# Autodesk Inventor assembly: Робот
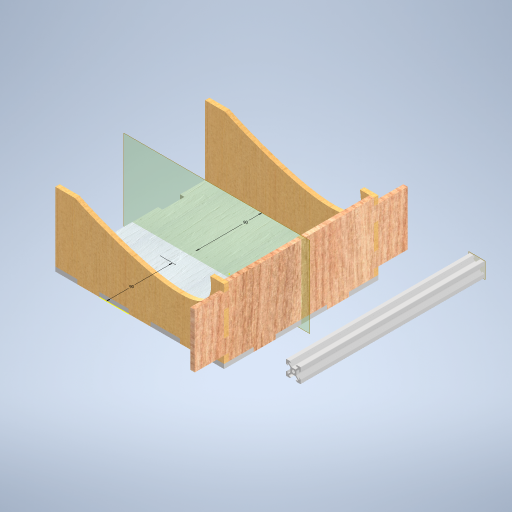
[picture p0: Inventor's stored thumbnail of the model, 512x512]
Saved by Autodesk Inventor 2024.2 (Build 282272000, 272)
## iProperties
Created: 2026-01-27
Part Number: Робот
Document SubType Name: Assembly
Designer: Service
Author: Service
## Documents named in this file (5)
- C:\Users\Zakhar\Documents\Artist-v2\3D\Робот.iam
- C:\Users\Zakhar\Documents\Artist-v2\3D\Низ робота.ipt
- C:\Users\Zakhar\Documents\Artist-v2\3D\бок.ipt
- C:\Users\Zakhar\Documents\Artist-v2\3D\перед.ipt
- C:\Users\Zakhar\Documents\Artist-v2\3D\в_профиль 2020.ipt
## Components (5 placed, 4 different names)
1. Низ робота:1 — Заподлицо:1, Совмещение:1, Заподлицо:2, Симметрия:1, Совмещение:2, Заподлицо:3, Заподлицо:4, Совмещение:3, Заподлицо:5
2. бок:1 — Заподлицо:1, Совмещение:1, Заподлицо:2, Симметрия:1
3. бок:2 — Совмещение:2, Заподлицо:3, Заподлицо:4
4. перед:1 — Совмещение:3, Заподлицо:5
5. в_профиль 2020:1
## Relationships (9: Flush 5, Mate 3, Symmetry 1)
- Заподлицо:1 [Flush]: Низ робота:1 ↔ бок:1
- Совмещение:1 [Mate]: Низ робота:1 ↔ бок:1
- Заподлицо:2 [Flush]: Низ робота:1 ↔ бок:1
- Симметрия:1 [Symmetry]: Низ робота:1 ↔ бок:1
- Совмещение:2 [Mate]: Низ робота:1 ↔ бок:2
- Заподлицо:3 [Flush]: Низ робота:1 ↔ бок:2
- Заподлицо:4 [Flush]: Низ робота:1 ↔ бок:2
- Совмещение:3 [Mate]: Низ робота:1 ↔ перед:1
- Заподлицо:5 [Flush]: Низ робота:1 ↔ перед:1
